# Autodesk Inventor assembly: WasabiV2
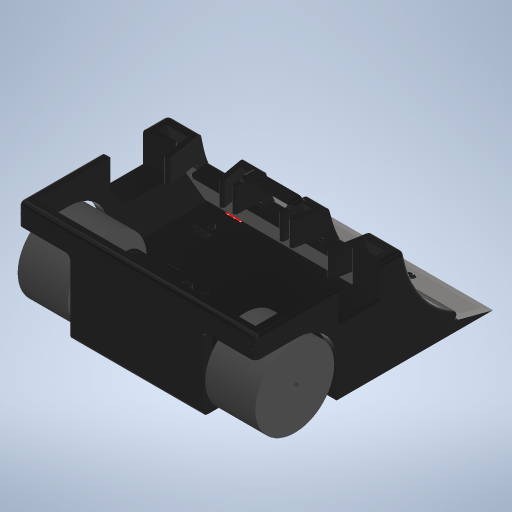
[picture p0: Inventor's stored thumbnail of the model, 512x512]
Saved by Autodesk Inventor 2024 (Build 280153000, 153)
## iProperties
Created: 2024-03-09
Part Number: WasabiV2
Document SubType Name: Assembly
Designer: kdcao
Author: kdcao
## Documents named in this file (6)
- C:\Users\kdcao\Documents\GitHub\wasabi2\Wasabi\WasabiV2.iam
- C:\Users\kdcao\Documents\GitHub\wasabi2\Wasabi\Body\bodyb2.ipt
- C:\Users\kdcao\Documents\GitHub\wasabi2\Wasabi\Bladev2.ipt
- C:\Users\kdcao\Documents\GitHub\wasabi2\Wasabi\Parts\micro-metal-gearmotor-standard.ipt
- C:\Users\kdcao\Documents\GitHub\wasabi2\Wasabi\Parts\wheel.ipt
- C:\Users\kdcao\Documents\GitHub\wasabi2\Wasabi\Parts\qtr-1a-reflectance-sensor.ipt
## Components (8 placed, 5 different names)
1. bodyb2:1 — Rotational:1, Rigid:1, Rigid:2, Rigid:3, Rigid:4
2. Bladev2:1 — Rotational:1
3. micro-metal-gearmotor-standard:1 — Rigid:2, Cylindrical:2
4. micro-metal-gearmotor-standard:2 — Rigid:1, Cylindrical:1
5. wheel:1 — Cylindrical:2
6. wheel:2 — Cylindrical:1
7. qtr-1a-reflectance-sensor:1 — Rigid:3
8. qtr-1a-reflectance-sensor:2 — Rigid:4
## Relationships (7: WeldJoint 4, CylindricalJoint 2, RevoluteJoint 1)
- Rotational:1 [RevoluteJoint]: bodyb2:1 ↔ Bladev2:1
- Rigid:1 [WeldJoint]: bodyb2:1 ↔ micro-metal-gearmotor-standard:2
- Rigid:2 [WeldJoint]: bodyb2:1 ↔ micro-metal-gearmotor-standard:1
- Cylindrical:1: micro-metal-gearmotor-standard:2 ↔ wheel:2
- Cylindrical:2: micro-metal-gearmotor-standard:1 ↔ wheel:1
- Rigid:3 [WeldJoint]: bodyb2:1 ↔ qtr-1a-reflectance-sensor:1
- Rigid:4 [WeldJoint]: bodyb2:1 ↔ qtr-1a-reflectance-sensor:2
